# Autodesk Inventor assembly: derive_base_plate_bottom_v6
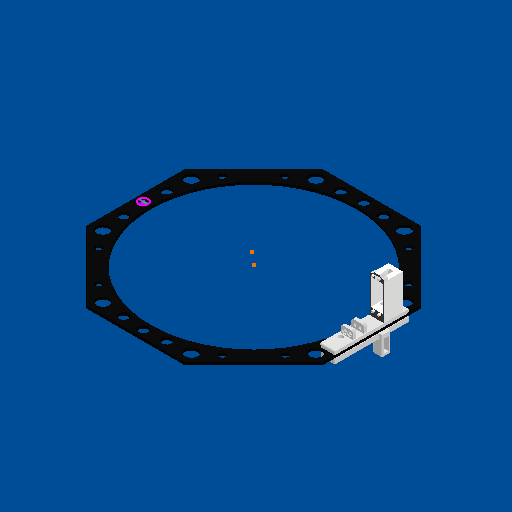
[picture p0: Inventor's stored thumbnail of the model, 512x512]
Saved by Autodesk Inventor 2026.2 (Build 302298000, 298)
## iProperties
Created: 2026-02-19
Part Number: derive_base_plate_bottom_v6
Document SubType Name: Assembly
Designer: Thoma
Author: Thoma
## Documents named in this file (4)
- C:\Users\Thoma\OneDrive\Desktop\dir\telescope_cover\cover\derive_base_plate_bottom_v6.iam
- C:\Users\Thoma\OneDrive\Desktop\dir\telescope_cover\cover\base_plate_bottom_v6.ipt
- C:\Users\Thoma\OneDrive\Desktop\dir\telescope_cover\telescope\version_4\Telescope_End.ipt
- C:\Users\Thoma\OneDrive\Desktop\dir\telescope_cover\cover\Base_plate_v15.ipt
## Components (3 placed, 3 different names)
1. base_plate_bottom_v6:1 — Mate:4, Flush:1, Flush:2
2. Telescope_End:1 — Mate:1, Mate:2, Mate:3, Mate:4
3. Base_plate_v15:1 — Mate:1, Mate:2, Mate:3, Flush:1, Flush:2
## Relationships (6: Mate 4, Flush 2)
- Mate:1: Telescope_End:1 ↔ Base_plate_v15:1
- Mate:2: Telescope_End:1 ↔ Base_plate_v15:1
- Mate:3: Telescope_End:1 ↔ Base_plate_v15:1
- Mate:4: base_plate_bottom_v6:1 ↔ Telescope_End:1
- Flush:1: base_plate_bottom_v6:1 ↔ Base_plate_v15:1
- Flush:2: base_plate_bottom_v6:1 ↔ Base_plate_v15:1
